# Autodesk Inventor assembly: przegub_3
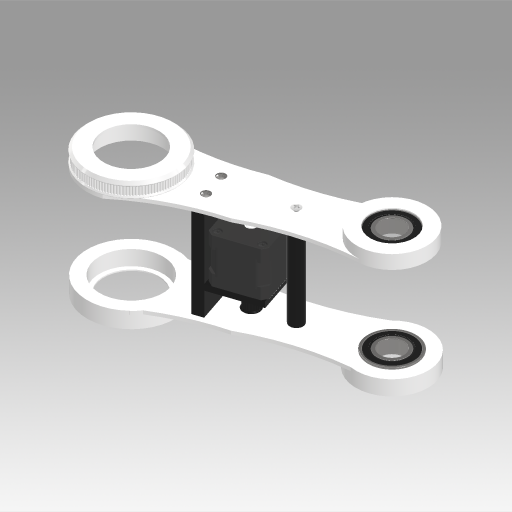
[picture p0: Inventor's stored thumbnail of the model, 512x512]
Saved by Autodesk Inventor 2024.3 (Build 283343000, 343)
## iProperties
Created: 2025-10-10
Part Number: przegub_3
Document SubType Name: Assembly
Designer: User
Mass: 262.129 g
Surface Area: 1421.84 cm^2
Volume: 262.129 cm^3
Author: User
## Documents named in this file (11)
- C:\Users\Duszy\Desktop\Dummy_v2\Model\Model\przegub_3\przegub_3.iam
- C:\Users\Duszy\Desktop\Dummy_v2\Model\Model\przegub_3\zebma.ipt
- C:\Users\Duszy\Desktop\Dummy_v2\Model\Model\przegub_3\20_zb_wal.ipt
- C:\Users\Duszy\Desktop\Dummy_v2\Model\Model\przegub_3\6661K87_Ball Bearing.ipt
- C:\Users\Duszy\Desktop\Dummy_v2\Model\Model\przegub_3\baza_rama3.ipt
- C:\Users\Duszy\Desktop\Dummy_v2\Model\Model\przegub_3\belkamid.ipt
- C:\Users\Duszy\Desktop\Dummy_v2\Model\Model\przegub_3\NEMA 17 Stepper Motor 39mm-NEMA 17 Stepper Motor 39mm.ipt
- C:\Users\Duszy\Desktop\Dummy_v2\Model\Model\przegub_3\os2_polatforma.ipt
- C:\Users\Duszy\Desktop\Dummy_v2\Model\Model\przegub_3\94459A774_Heat-Set Inserts for Plastic.ipt
- C:\Users\Duszy\Desktop\Dummy_v2\Model\Model\przegub_3\m4-10mm_bc.ipt
- C:\Users\Duszy\Desktop\Dummy_v2\Model\Model\przegub_3\m3-10mm_bc.ipt
## Components (24 placed, 10 different names)
1. zebma:1 — Obrotowe:6, Obrotowe:7, Obrotowe:10
2. 20_zb_wal:1 — Obrotowe:2
3. 6661K87_Ball Bearing:1 — Obrotowe:8
4. baza_rama3:1 — Obrotowe:8, Sztywne:7
5. belkamid:1 — Obrotowe:9, Sztywne:6
6. NEMA 17 Stepper Motor 39mm-NEMA 17 Stepper Motor 39mm:1 — Obrotowe:1, Obrotowe:11, Obrotowe:2
7. os2_polatforma:1 — Obrotowe:11, Obrotowe:3, Obrotowe:4, Obrotowe:6, Sztywne:7
8. 6661K87_Ball Bearing:2 — Obrotowe:7
9. m4-10mm_bc:1 — Sztywne:2
10. 94459A774_Heat-Set Inserts for Plastic:2 — Sztywne:2, Obrotowe:9, Obrotowe:10
11. m4-10mm_bc:6
12. 94459A774_Heat-Set Inserts for Plastic:7 — Sztywne:6
13. m3-10mm_bc:1 — Obrotowe:1
14. m3-10mm_bc:2
15. m3-10mm_bc:3
16. m3-10mm_bc:4
17. m4-10mm_bc:2
18. 94459A774_Heat-Set Inserts for Plastic:3 — Obrotowe:3
19. m4-10mm_bc:4
20. 94459A774_Heat-Set Inserts for Plastic:5
21. 94459A774_Heat-Set Inserts for Plastic:4 — Obrotowe:4
22. m4-10mm_bc:3
23. 94459A774_Heat-Set Inserts for Plastic:6
24. m4-10mm_bc:5
## Component patterns: (4 elements, first: m3-10mm_bc:1), (2 elements, first: m4-10mm_bc:2 + 94459A774_Heat-Set Inserts for Plastic:3), (2 elements, first: 94459A774_Heat-Set Inserts for Plastic:4 + m4-10mm_bc:3)
## Relationships (16: RevoluteJoint 10, WeldJoint 6)
- Obrotowe:1 [RevoluteJoint] (-3 mm): NEMA 17 Stepper Motor 39mm-NEMA 17 Stepper Motor 39mm:1 ↔ m3-10mm_bc:1
- Obrotowe:11 [RevoluteJoint] (-5 mm): NEMA 17 Stepper Motor 39mm-NEMA 17 Stepper Motor 39mm:1 ↔ os2_polatforma:1
- Obrotowe:2 [RevoluteJoint]: 20_zb_wal:1 ↔ NEMA 17 Stepper Motor 39mm-NEMA 17 Stepper Motor 39mm:1
- Sztywne:2 [WeldJoint] (-5 mm): m4-10mm_bc:1 ↔ 94459A774_Heat-Set Inserts for Plastic:2
- [WeldJoint] (-6 mm): m4-10mm_bc:2 ↔ 94459A774_Heat-Set Inserts for Plastic:3
- Obrotowe:3 [RevoluteJoint]: os2_polatforma:1 ↔ 94459A774_Heat-Set Inserts for Plastic:3
- [WeldJoint] (-6 mm): 94459A774_Heat-Set Inserts for Plastic:4 ↔ m4-10mm_bc:3
- Obrotowe:4 [RevoluteJoint]: os2_polatforma:1 ↔ 94459A774_Heat-Set Inserts for Plastic:4
- Obrotowe:6 [RevoluteJoint]: zebma:1 ↔ os2_polatforma:1
- Obrotowe:7 [RevoluteJoint] (-10 mm): zebma:1 ↔ 6661K87_Ball Bearing:2
- Obrotowe:8 [RevoluteJoint] (-10 mm): 6661K87_Ball Bearing:1 ↔ baza_rama3:1
- Obrotowe:9 [RevoluteJoint]: belkamid:1 ↔ 94459A774_Heat-Set Inserts for Plastic:2
- [WeldJoint] (-5 mm): m4-10mm_bc:6 ↔ 94459A774_Heat-Set Inserts for Plastic:7
- Sztywne:6 [WeldJoint]: belkamid:1 ↔ 94459A774_Heat-Set Inserts for Plastic:7
- Obrotowe:10 [RevoluteJoint]: zebma:1 ↔ 94459A774_Heat-Set Inserts for Plastic:2
- Sztywne:7 [WeldJoint] (3 mm): baza_rama3:1 ↔ os2_polatforma:1
## Named parameters: d8_d7 = -6 mm, d11_d7 = -6 mm, d36_d7 = -5 mm
